# Autodesk Inventor assembly: Fanwithscrews
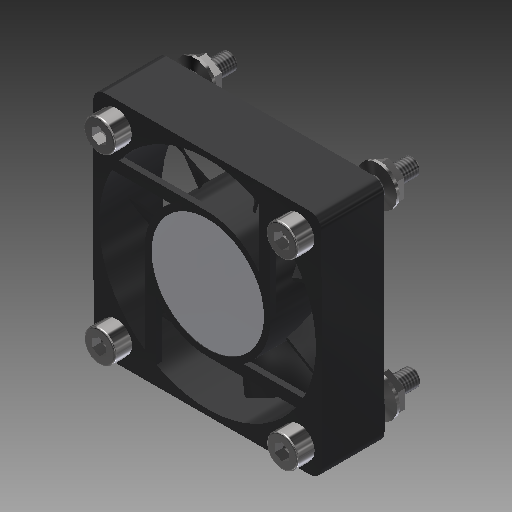
[picture p0: Inventor's stored thumbnail of the model, 512x512]
Saved by Autodesk Inventor 2017 (Build 210142000, 142)
## iProperties
Created: 2016-07-28
Part Number: Fanwithscrews
Document SubType Name: Assembly
Designer: User
Author: User
## Documents named in this file (5)
- C:\All INVENTOR\SL-Inventor\SL-Beast 3D Printer\Fanwithscrews.iam
- C:\All INVENTOR\SL-Inventor\SL-Beast 3D Printer\40mm_fan_MIR.ipt
- C:\All INVENTOR\SL-Inventor\SL-Beast 3D Printer\en-US\ANSI B18.3.1M(6)\ANSI B18.3.1M - M3x0.5 x 20(1).ipt
- C:\All INVENTOR\SL-Inventor\SL-Beast 3D Printer\en-US\JIS B 1251 C1 (1L 1H)\JIS B 1251  - 3 1L.ipt
- C:\All INVENTOR\SL-Inventor\SL-Beast 3D Printer\en-US\CSN EN 24 036\CSN EN 24 036 - M3.ipt
## Components (13 placed, 4 different names)
1. 40mm_fan_MIR:1
2. Forged Socket Head Cap Screw - Metric M3x0.5 x 20:1
3. Forged Socket Head Cap Screw - Metric M3x0.5 x 20:2
4. Forged Socket Head Cap Screw - Metric M3x0.5 x 20:3
5. Forged Socket Head Cap Screw - Metric M3x0.5 x 20:4
6. JIS B 1251 Class 1 (1L/1H) 3 1L:1
7. JIS B 1251 Class 1 (1L/1H) 3 1L:2
8. JIS B 1251 Class 1 (1L/1H) 3 1L:3
9. JIS B 1251 Class 1 (1L/1H) 3 1L:4
10. CSN EN 24036 M3:1
11. CSN EN 24036 M3:2
12. CSN EN 24036 M3:3
13. CSN EN 24036 M3:4
## Relationships (12: Mate 8, Insert 4)
- [Insert]: 40mm_fan_MIR:1 ↔ Forged Socket Head Cap Screw - Metric M3x0.5 x 20:1
- [Insert]: 40mm_fan_MIR:1 ↔ Forged Socket Head Cap Screw - Metric M3x0.5 x 20:2
- [Insert]: 40mm_fan_MIR:1 ↔ Forged Socket Head Cap Screw - Metric M3x0.5 x 20:3
- [Insert]: 40mm_fan_MIR:1 ↔ Forged Socket Head Cap Screw - Metric M3x0.5 x 20:4
- [Mate]: Forged Socket Head Cap Screw - Metric M3x0.5 x 20:1 ↔ JIS B 1251 Class 1 (1L/1H) 3 1L:1
- [Mate]: Forged Socket Head Cap Screw - Metric M3x0.5 x 20:3 ↔ JIS B 1251 Class 1 (1L/1H) 3 1L:2
- [Mate]: Forged Socket Head Cap Screw - Metric M3x0.5 x 20:2 ↔ JIS B 1251 Class 1 (1L/1H) 3 1L:3
- [Mate]: Forged Socket Head Cap Screw - Metric M3x0.5 x 20:4 ↔ JIS B 1251 Class 1 (1L/1H) 3 1L:4
- [Mate]: Forged Socket Head Cap Screw - Metric M3x0.5 x 20:1 ↔ CSN EN 24036 M3:1
- [Mate]: Forged Socket Head Cap Screw - Metric M3x0.5 x 20:3 ↔ CSN EN 24036 M3:2
- [Mate]: Forged Socket Head Cap Screw - Metric M3x0.5 x 20:4 ↔ CSN EN 24036 M3:3
- [Mate]: Forged Socket Head Cap Screw - Metric M3x0.5 x 20:2 ↔ CSN EN 24036 M3:4
